(part 1 of 3)
# Autodesk Inventor assembly: 000 Ensamblaje hw_LM - BASIC
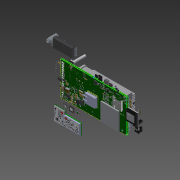
[picture p0: Inventor's stored thumbnail of the model, 180x180]
Saved by Autodesk Inventor 2018 (Build 220112000, 112)
## iProperties
Created: 2025-09-15
Part Number: 000 Ensamblaje hw_LM - BASIC
Document SubType Name: Assembly
Designer: mbs18
Author: mbs18
## Documents named in this file (68)
- C:\Users\mbs18.Embention\Git\LM\items\3d_LM\hw_LM\3d\000 Ensamblaje hw_LM - BASIC.iam
- C:\Users\mbs18.Embention\Git\LM\items\3d_LM\hw_LM\3d\hw_LM - PCB.ipt
- C:\Users\mbs18.Embention\Git\LM\items\_accesories\Cables y conectores\3d_Te Connectivity\3d\2309413-1\2309413-1.ipt
- C:\Users\mbs18.Embention\Git\LM\items\_accesories\Componentes PCB\Jetson Orin Nano\Nvidia\Jetson_Orin_NX_Orin_Nano_Module_3D_STEP_Model_20230310\P3767-pcba-envelop_20230310.ipt
- C:\Users\mbs18.Embention\Git\LM\items\_accesories\Componentes PCB\Tarjetero\3d_Molex\3d\47219-2001.ipt
- C:\Users\mbs18.Embention\Git\LM\items\_accesories\Componentes PCB\Magnetometro\3d_PNI Corp\3d\RM3100\Sen-XY-f.ipt
- C:\Users\mbs18.Embention\Git\LM\items\_accesories\Componentes PCB\Magnetometro\3d_PNI Corp\3d\RM3100\Sen-Z-f.ipt
- C:\Users\mbs18.Embention\Git\LM\items\_accesories\Componentes PCB\Transformadores de señal\3d_Pulse_Electronics\HX5008NL\HX5008NL.iam
- C:\Users\mbs18.Embention\Git\LM\items\_accesories\Componentes PCB\Conectores\3d_Samtec\3d\CLP-104-02-F-D-BE-TR.ipt
- C:\Users\mbs18.Embention\Git\LM\items\_accesories\Componentes PCB\Magnetometro\3d_PNI Corp\3d\RM3100\MAGI2C.ipt
- C:\Users\mbs18.Embention\Git\LM\items\_accesories\Componentes PCB\Inductor\3d_Vishay\IHLP2020CZER2R2MA1\IHLP2020CZER1R0M01.ipt
- C:\Users\mbs18.Embention\Git\LM\items\_accesories\Componentes PCB\Capacitadores\3d_Kemet\3d\CL31B106KBK6PJE.ipt
- C:\Users\mbs18.Embention\Git\LM\items\_accesories\Componentes PCB\Resistencias\3d_Genérico\R0805.ipt
- C:\Users\mbs18.Embention\Git\LM\items\_accesories\Componentes PCB\Resistencias\3d_Mouser Electronics\3d\ERJ-U02F1601X\RES-1.6K_1%_0402.iam
- C:\Users\mbs18.Embention\Git\LM\items\_accesories\Componentes PCB\Conversores\CC-CC\3d_MuRata\3d\3d_MGJ1D121505MPC-R7\UND_0201CR___ _________.ipt
- C:\Users\mbs18.Embention\Git\LM\items\_accesories\Componentes PCB\Led\3d_ROHM EXCELED\3d\SML-D12V8WT86C.ipt
- C:\Users\mbs18.Embention\Git\LM\items\_accesories\Componentes PCB\IMU\3d_Bosch\3d\BMI088.ipt
- C:\Users\mbs18.Embention\Git\LM\items\_accesories\Componentes PCB\Reguladores\3d_Texas Instruments\3d\TPS7A5301QRGRRQ1\TPS7A5301QRGRRQ1.iam
- C:\Users\mbs18.Embention\Git\LM\items\_accesories\Componentes PCB\Ferrita\3d_Murata Electronics\3d\BLM21PG220SN1D.ipt
- C:\Users\mbs18.Embention\Git\LM\items\_accesories\Componentes PCB\Condensadores\3d_KEMET\3d\C0603C101K5GAC3190\C0603C101K5GAC3190.ipt
- C:\Users\mbs18.Embention\Git\LM\items\_accesories\Componentes PCB\Capacitadores\3d_Kemet\3d\C1206C152KGRACAUTO.ipt
- C:\Users\mbs18.Embention\Git\LM\items\_accesories\Componentes PCB\Diodos\3d_Littlefuse\3d\AQ24CANFD-02HTG.ipt
- C:\Users\mbs18.Embention\Git\LM\items\_accesories\Componentes PCB\Oscilador\3d_ECS_International\ECS-2520MVQ-250-CN-TR\ECS-2520MVQ-250-CN-TR.ipt
- C:\Users\mbs18.Embention\Git\LM\items\_accesories\Componentes PCB\Jetson Orin Nano\Nvidia\Jetson_Orin_Nano_DevKit_3D_STEP_Model\095-0180-000-TS1_ASM.iam
- C:\Users\mbs18.Embention\Git\LM\items\_accesories\Componentes PCB\Microcontroladores\S32E288ABCAAMJGT.ipt
- C:\Users\mbs18.Embention\Git\LM\items\_accesories\Componentes PCB\Transceptor\3d_Texas Instrument\3d\DP83867ERGZT\DP83867ERGZT.iam
- C:\Users\mbs18.Embention\Git\LM\items\_accesories\Componentes PCB\DC-DC\3d_Linear Technology\3d\LTC7103IUHE#PBF.ipt
- C:\Users\mbs18.Embention\Git\LM\items\_accesories\Componentes PCB\CAN\3d\3d_Texas_Instruments\TCAN1462VDRBRQ1\TCAN1462VDRBRQ1.iam
- C:\Users\mbs18.Embention\Git\LM\items\_accesories\Componentes PCB\Mosfet\3d_Vishay\3d\SQJ465EP-T1_GE3\SQJ465EP-T1_GE3.iam
- C:\Users\mbs18.Embention\Git\LM\items\_accesories\Componentes PCB\Capacitadores\3d_Kyocera\3d\KAM55CR72A106KV-C2220K-simpl.ipt
- C:\Users\mbs18.Embention\Git\LM\items\_accesories\Componentes PCB\Schottky Diodes\3d_STMicroelectronics\3d\STPS5H100AFY\STPS5H100AFY.ipt
- C:\Users\mbs18.Embention\Git\LM\items\_accesories\Componentes PCB\Diodos\3d_Bourns\3d\SMA6J64CA\SMA6J64CA.ipt
- C:\Users\mbs18.Embention\Git\LM\items\_accesories\Componentes PCB\Condensadores\3d_KEMET\3d\C1210C472KGRACAUTO\C1210C472KGRACAUTO.ipt
- C:\Users\mbs18.Embention\Git\LM\items\_accesories\Componentes PCB\Mosfet\3d_Infineon\3d\BSS123NH6327XTSA1\BSS123NH6327XTSA1.iam
- C:\Users\mbs18.Embention\Git\LM\items\_accesories\Componentes PCB\Diodos\3d_Vishay\3d\BZD27C10P-HE3-08.ipt
- C:\Users\mbs18.Embention\Git\LM\items\_accesories\Componentes PCB\Condensadores\3d_KEMET\3d\C0603C103K1RECAUTO\C0603C103K1RECAUTO.iam
- C:\Users\mbs18.Embention\Git\LM\items\_accesories\Componentes PCB\DC-DC\3d_Texas Instruments\3d\LM5146QRGYRQ1\LM5146QRGYRQ1.iam
- C:\Users\mbs18.Embention\Git\LM\items\_accesories\Componentes PCB\Bobinas\3d_COILCRAFT\3d\1812CAN-113NRC\1812CAN-113NRC.iam
- C:\Users\mbs18.Embention\Git\LM\items\_accesories\Componentes PCB\Diodos\3d_ST Microelectronics\HSP051-4M10\HSP051-4M10.ipt
- C:\Users\mbs18.Embention\Git\LM\items\_accesories\Componentes PCB\IMU\3d_Analog Devices\3d\ADIS16505-3BMLZ\ADIS16505-3BMLZ.ipt
- C:\Users\mbs18.Embention\Git\LM\items\_accesories\Componentes PCB\SIM\3d_EMNIFY\3d\ESIM 638037665970.ipt
- C:\Users\mbs18.Embention\Git\LM\items\_accesories\Componentes PCB\CAN\3d\Analog Devices\LTC2875MPDD#PBF.ipt
- C:\Users\mbs18.Embention\Git\LM\items\_accesories\Componentes PCB\Transceptor\3d_Texas Instrument\3d\UQFN-16.ipt
- C:\Users\mbs18.Embention\Git\LM\items\_accesories\Componentes PCB\Oscilador\3d_ECS_International\ECS-400-8-33Q-ADS-TR.ipt
- C:\Users\mbs18.Embention\Git\LM\items\_accesories\Componentes PCB\DC-DC\3d_Texas Instruments\3d\TPS3897ADRYT.ipt
- C:\Users\mbs18.Embention\Git\LM\items\_accesories\Componentes PCB\ESD Protection\3d_Nexperia\3d\PESD2CANFD27V-UX\PESD2CANFD27V-UX.iam
- C:\Users\mbs18.Embention\Git\LM\items\_accesories\Componentes PCB\Diodos\3d_Diodes Incorporated\3d\DMN2710UTQ-7\DMN2710UTQ-7.ipt
- C:\Users\mbs18.Embention\Git\LM\items\_accesories\Componentes PCB\Multiplexor\3d_TI\3d\SN74LVC1G08QDCKRQ1.ipt
- C:\Users\mbs18.Embention\Git\LM\items\_accesories\Cables y conectores\3d_Molex\3d\53398-0471.ipt
- C:\Users\mbs18.Embention\Git\LM\items\_accesories\Componentes PCB\Bobinas\3d_COILCRAFT\3d\XAL7030-472MEC\XAL7030-472MEC.iam
- C:\Users\mbs18.Embention\Git\LM\items\_accesories\Componentes PCB\Mosfet\3d_Vishay\3d\SQJ402EP-T1_GE3.ipt
- C:\Users\mbs18.Embention\Git\LM\items\_accesories\Componentes PCB\Resistencias\3d_Genérico\MMB02070B1007GB200.ipt
- C:\Users\mbs18.Embention\Git\LM\items\_accesories\Componentes PCB\Inductor\3d_TDK\3d\XAL4020-601MEC\XAL4020-601MEC.ipt
- C:\Users\mbs18.Embention\Git\LM\items\_accesories\Componentes PCB\Reguladores\3d_Analog\3d\LTC3310SIV#PBF.ipt
- C:\Users\mbs18.Embention\Git\LM\items\_accesories\Componentes PCB\Diodos\3d_Texas Instrument\3d\TPD4E05U06QDQARQ1.ipt
- C:\Users\mbs18.Embention\Git\LM\items\_accesories\Componentes PCB\Diodos\3d_Littlefuse\3d\AQ05C-01FTG\AQ05C-01FTG.ipt
- C:\Users\mbs18.Embention\Git\LM\items\_accesories\Componentes PCB\GSM\3d_U-blox\3d\Sara\SARA.iam
- C:\Users\mbs18.Embention\Git\LM\items\_accesories\Componentes PCB\GPS - GNSS\3d_U-blox\3d\ZED F9P\u-blox ZED-F9P.ipt
- C:\Users\mbs18.Embention\Git\LM\items\_accesories\Componentes PCB\Elementos mecanicos soldables\3d_Wurth Electronics\3d\9774065151.ipt
- C:\Users\mbs18.Embention\Git\LM\items\_accesories\Ordenadores y Tablets\3d_NVIDIA\3d\Orin nano\Heatsink\ATS-NVP-3281-C2-R0.ipt
- C:\Users\mbs18.Embention\Git\LM\items\_accesories\Componentes PCB\Elementos mecanicos soldables\3d_Wurth Electronics\3d\9774130960R.ipt
- C:\Users\mbs18.Embention\Git\LM\items\_accesories\Sensores\Sensor de presion\3d_Amphenol\3d\AUAV-L10D-M25125-RR-N.ipt
- C:\Users\mbs18.Embention\Git\LM\items\_accesories\Componentes PCB\Resistencias\3d_Genérico\RESC-1210.ipt
- C:\Users\mbs18.Embention\Git\LM\items\_accesories\Componentes PCB\Reguladores\3d_Analog\3d\LIB_LTC7103MPUHE#PBF\LTC7103MPUHE#PBF.ipt
- C:\Users\mbs18.Embention\Git\LM\items\_accesories\Componentes PCB\Active-low load\3d_Texas_Instruments\TPS22910AYZVR\Body.ipt
- C:\Users\mbs18.Embention\Git\LM\items\_accesories\Componentes PCB\Led\3d_Lumex\3d\LPA-C011301S.ipt
- C:\Users\mbs18.Embention\Git\LM\items\_accesories\Componentes PCB\Sensores de Presion\3d_TE Connectivity\3d\MS561101BA03-50.ipt
- C:\Users\mbs18.Embention\Git\LM\items\_accesories\Componentes PCB\Sensores de Presion\3d_Infineon\3d\DPS368XTSA1.ipt
## Components (484 placed, 67 different names)
1. hw_LM - PCB:1 — Mate:1, Flush:1, Flush:2, Mate:4, Mate:29, Angle:6, Mate:33, Mate:35, Mate:47, Mate:58, Mate:59, Mate:60, Mate:69, Mate:72, Mate:73, Mate:81, Mate:83, Mate:84, Mate:94, Mate:95, Mate:96, Mate:97, Mate:98, Angle:44, Mate:99, Mate:100, Mate:101, Mate:102, Angle:45, Mate:103, Mate:104, Mate:105, Mate:107, Mate:108, Mate:109, Mate:110, Mate:112, Mate:113, Mate:114, Mate:115, Mate:116, Mate:117, Mate:118, Angle:49, Angle:50, Mate:119, Mate:120, Mate:121, Angle:53, Mate:122, Mate:123, Mate:124, Mate:125, Mate:126, Mate:127, Mate:128, Mate:129, Mate:130, Mate:131, Mate:132, Angle:59, Mate:133, Mate:134, Angle:62, Mate:135, Angle:64, Mate:136, Angle:86, Mate:137, Mate:138, Mate:139, Mate:140, Angle:88, Mate:141, Mate:142, Mate:143, Mate:144, Mate:145, Tangent:1, Mate:146, Mate:147, Mate:148, Mate:149, Mate:150, Mate:151, Mate:152, Mate:153, Mate:154, Mate:155, Angle:91, Mate:158, Angle:134, Angle:135, Mate:159, Mate:163, Mate:165, Mate:167, Mate:182, Mate:184, Mate:185, Mate:186, Mate:187, Mate:188, Mate:189, Mate:190, Mate:191, Mate:192, Mate:193
2. 095-0180-000-TS1_ASM:1 [sub-assembly]
3. 2309413-1:1 — Mate:4, Mate:58, Mate:59
4. P3767-pcba-envelop_20230310:1 — Mate:154, Mate:155, Mate:163, Mate:164, Mate:166, Mate:168, Mate:169, Mate:170, Mate:171
5. 47219-2001:1 — Mate:29, Angle:6
6. Sen-XY-f:1 — Mate:35, Flush:16
7. Sen-Z-f:1 — Mate:33
8. Sen-XY-f:2 — Flush:16
9. CLP-104-02-F-D-BE-TR:1 — Mate:47
10. HX5008NL:3 [sub-assembly] — Mate:83
11. HX5008NL:4 [sub-assembly] — Angle:44, Mate:99
12. MAGI2C:1 — Mate:60
13. IHLP2020CZER1R0M01:2
14. R0805:1 — Mate:69, Flush:39, Flush:40
15. R0805:2 — Flush:39
16. R0805:3 — Flush:40
17. CL31B106KBK6PJE:7 — Flush:43
18. CL31B106KBK6PJE:8 — Flush:43
19. UND_0201CR___ _________:1 — Mate:73, Flush:44
20. UND_0201CR___ _________:2 — Flush:44
21. BLM21PG220SN1D:4
22. C0603C101K5GAC3190:6 — Flush:119, Angle:56
23. C0603C101K5GAC3190:7 — Flush:119, Angle:56
24. BLM21PG220SN1D:11
25. C1206C152KGRACAUTO:1 — Mate:81, Flush:124, Angle:49
26. C1206C152KGRACAUTO:2 — Flush:123, Flush:124, Angle:48
27. C1206C152KGRACAUTO:3 — Flush:122, Flush:123, Flush:221, Flush:222, Flush:432
28. C1206C152KGRACAUTO:4 — Flush:122, Angle:48
29. BLM21PG220SN1D:12 — Flush:125
30. BLM21PG220SN1D:13 — Flush:125, Flush:126
31. BLM21PG220SN1D:14 — Flush:126, Flush:127
32. BLM21PG220SN1D:15 — Flush:127
33. AQ24CANFD-02HTG:5
34. AQ24CANFD-02HTG:6
35. AQ24CANFD-02HTG:7
36. AQ24CANFD-02HTG:8
37. S32E288ABCAAMJGT:1 — Mate:94, Angle:58, Angle:60, Angle:141
38. DP83867ERGZT:1 [sub-assembly] — Mate:95, Angle:43
39. ECS-2520MVQ-250-CN-TR:2 — Mate:96, Angle:43
40. LTC7103IUHE#PBF:1 — Mate:97
41. TCAN1462VDRBRQ1:1 [sub-assembly] — Mate:98, Flush:201
42. TCAN1462VDRBRQ1:2 [sub-assembly] — Flush:200
43. TCAN1462VDRBRQ1:3 [sub-assembly] — Flush:200, Flush:201
44. SQJ465EP-T1_GE3:1 [sub-assembly] — Mate:100, Mate:101
45. KAM55CR72A106KV-C2220K-simpl:1 — Mate:102, Angle:45, Angle:46, Angle:47
46. KAM55CR72A106KV-C2220K-simpl:2 — Mate:103, Angle:110
47. STPS5H100AFY:1 — Mate:104, Angle:46
48. STPS5H100AFY:3 — Mate:105, Angle:109
49. SML-D12V8WT86C:2 — Mate:107, Flush:202, Flush:611
50. SML-D12V8WT86C:3 — Mate:108
51. SML-D12V8WT86C:4 — Mate:109
52. SML-D12V8WT86C:5 — Mate:110
53. SML-D12V8WT86C:6 — Flush:202
54. SMA6J64CA:1 — Mate:116, Angle:47, Angle:63
55. SMA6J64CA:2 — Mate:117
56. C1210C472KGRACAUTO:1 — Mate:118, Flush:211
57. C1210C472KGRACAUTO:2 — Flush:210, Flush:211
58. C1210C472KGRACAUTO:3 — Flush:210
59. BSS123NH6327XTSA1:1 [sub-assembly] — Angle:50, Mate:119
60. BZD27C10P-HE3-08:1 — Mate:120
61. C0603C103K1RECAUTO:1 [sub-assembly] — Mate:121, Flush:217, Flush:219, Flush:335
62. C0603C103K1RECAUTO:2 [sub-assembly] — Flush:213, Flush:214
63. C0603C103K1RECAUTO:3 [sub-assembly] — Flush:218
64. C0603C103K1RECAUTO:4 [sub-assembly] — Flush:215
65. C0603C103K1RECAUTO:5 [sub-assembly] — Flush:212, Flush:213, Flush:216, Flush:217
66. C0603C103K1RECAUTO:6 [sub-assembly] — Flush:212, Flush:215, Flush:337
67. C0603C103K1RECAUTO:7 [sub-assembly] — Flush:214, Flush:427
68. C0603C103K1RECAUTO:8 [sub-assembly] — Flush:216, Flush:218, Flush:219
69. C0603C103K1RECAUTO:9 [sub-assembly] — Angle:53, Flush:222, Flush:223
70. C0603C103K1RECAUTO:10 [sub-assembly] — Flush:221
71. C0603C103K1RECAUTO:11 [sub-assembly] — Flush:223
72. C1210C472KGRACAUTO:7 — Flush:224
73. C1210C472KGRACAUTO:8 — Flush:224, Flush:231
74. LM5146QRGYRQ1:1 [sub-assembly] — Mate:122, Angle:76
75. 1812CAN-113NRC:1 [sub-assembly] — Mate:123
76. TCAN1462VDRBRQ1:5 [sub-assembly] — Mate:124
77. C1210C472KGRACAUTO:9 — Flush:229, Flush:231
78. C1210C472KGRACAUTO:10 — Flush:229
79. C1210C472KGRACAUTO:11 — Flush:228, Flush:230, Flush:232
80. C1210C472KGRACAUTO:12 — Flush:228, Flush:230, Flush:232, Angle:65
81. HSP051-4M10:1 — Mate:126, Flush:330, Flush:332
82. HSP051-4M10:2 — Flush:330
83. ADIS16505-3BMLZ:1 — Mate:127
84. BMI088:2 — Mate:128
85. ESIM 638037665970:1 — Mate:129, Angle:58
86. TPS7A5301QRGRRQ1:2 [sub-assembly] — Mate:130
87. LTC2875MPDD#PBF:1 — Mate:131, Flush:331
88. UQFN-16:1 — Mate:132, Angle:59
89. LTC2875MPDD#PBF:2 — Flush:331
90. ECS-400-8-33Q-ADS-TR:1 — Mate:133, Angle:60
91. TPS3897ADRYT:1 — Mate:134
92. HSP051-4M10:3 — Flush:332
93. PESD2CANFD27V-UX:1 [sub-assembly] — Angle:62, Mate:135, Angle:63
94. DMN2710UTQ-7:1 — Angle:64, Mate:136, Angle:65, Flush:333
95. DMN2710UTQ-7:2 — Flush:333, Flush:338
96. C0603C103K1RECAUTO:12 [sub-assembly] — Flush:334
97. C0603C103K1RECAUTO:13 [sub-assembly] — Flush:334, Flush:335
98. C0603C103K1RECAUTO:14 [sub-assembly] — Flush:336, Flush:337
99. C0603C103K1RECAUTO:15 [sub-assembly] — Flush:336
100. DMN2710UTQ-7:3 — Flush:339, Flush:340
101. DMN2710UTQ-7:4 — Flush:338, Flush:339, Flush:422
102. DMN2710UTQ-7:5 — Flush:340
103. DMN2710UTQ-7:6 — Flush:601
104. DMN2710UTQ-7:7 — Flush:422, Flush:423, Flush:603
105. DMN2710UTQ-7:8 — Flush:423
106. SN74LVC1G08QDCKRQ1:1 — Angle:86, Mate:137, Flush:602
107. C0603C103K1RECAUTO:16 [sub-assembly] — Flush:424, Flush:426, Flush:427
108. C0603C103K1RECAUTO:17 [sub-assembly] — Flush:425, Flush:426, Flush:431
109. C0603C103K1RECAUTO:18 [sub-assembly] — Flush:424
110. C0603C103K1RECAUTO:19 [sub-assembly] — Flush:425
111. C0603C103K1RECAUTO:20 [sub-assembly]
112. C0603C103K1RECAUTO:21 [sub-assembly] — Flush:431
113. C0603C103K1RECAUTO:22 [sub-assembly]
114. C0603C103K1RECAUTO:23 [sub-assembly]
115. UQFN-16:2 — Mate:138, Angle:141
116. C1206C152KGRACAUTO:5 — Flush:432
117. 53398-0471:1 — Mate:140, Angle:88
118. XAL7030-472MEC:1 [sub-assembly] — Mate:141, Flush:433
119. XAL7030-472MEC:2 [sub-assembly] — Flush:433
120. SQJ402EP-T1_GE3:1 — Mate:142, Mate:143
121. SQJ402EP-T1_GE3:2 — Mate:144, Mate:145
122. MMB02070B1007GB200:1 — Tangent:1
123. C1210C472KGRACAUTO:13 — Mate:146
124. C1206C152KGRACAUTO:6 — Mate:147
125. C1206C152KGRACAUTO:7 — Flush:436
126. C1206C152KGRACAUTO:8 — Flush:436
127. R0805:4 — Mate:148, Flush:437, Flush:440, Flush:443
128. R0805:5 — Flush:438, Flush:439
129. R0805:6 — Flush:439, Flush:440
130. R0805:7 — Flush:437, Flush:438
131. R0805:8
132. R0805:9
133. R0805:10 — Flush:443
134. 1812CAN-113NRC:2 [sub-assembly] — Mate:149
135. XAL4020-601MEC:1 — Mate:150, Flush:444
136. XAL4020-601MEC:2 — Flush:444
137. XAL4020-601MEC:3 — Mate:188
138. BZD27C10P-HE3-08:2 — Mate:151
139. LTC3310SIV#PBF:1 — Mate:152, Flush:446
140. LTC3310SIV#PBF:2 — Flush:446
141. TPD4E05U06QDQARQ1:1 — Mate:153, Flush:447
142. TPD4E05U06QDQARQ1:2 — Flush:448
143. TPD4E05U06QDQARQ1:3 — Flush:447, Flush:448
144. PESD2CANFD27V-UX:2 [sub-assembly] — Mate:158, Angle:109, Flush:536
145. PESD2CANFD27V-UX:3 [sub-assembly] — Flush:536, Angle:110
146. AQ05C-01FTG:1 — Angle:134, Angle:135, Mate:159
147. u-blox ZED-F9P:1 — Mate:185, Angle:137
148. 9774065151:1 — Mate:164, Mate:165
149. 9774065151:2 — Mate:166, Mate:167
150. ATS-NVP-3281-C2-R0:1 — Mate:168, Mate:169, Mate:170, Mate:171
151. AUAV-L10D-M25125-RR-N:1 — Mate:182, Angle:139
152. SARA:1 [sub-assembly] — Mate:184, Angle:138
153. DMN2710UTQ-7:9 — Flush:601
154. SN74LVC1G08QDCKRQ1:2 — Flush:602
155. DMN2710UTQ-7:10 — Flush:603
156. RESC-1210:1 — Mate:186, Angle:137
157. LTC7103MPUHE#PBF:1 — Mate:187, Angle:138
158. C1210C472KGRACAUTO:14 — Mate:189, Angle:139, Flush:605, Flush:609
159. C1210C472KGRACAUTO:15 — Flush:604, Flush:605, Flush:608
160. C1210C472KGRACAUTO:16 — Flush:604, Flush:606, Flush:607
161. C1210C472KGRACAUTO:17 — Flush:606, Flush:608
162. C1210C472KGRACAUTO:18 — Flush:607
163. C1210C472KGRACAUTO:19
164. C1210C472KGRACAUTO:20 — Flush:610
165. C1210C472KGRACAUTO:21 — Flush:609, Flush:610
166. Body:1 — Mate:190
167. LPA-C011301S:1 — Mate:191
168. SML-D12V8WT86C:7 — Flush:611
169. MS561101BA03-50:1 — Mate:192, Angle:140
170. DPS368XTSA1:1 — Mate:193
171. 9774130960R:1
172. RES-1.6K_1%_0402:263 [sub-assembly] — Angle:95, Flush:517, Flush:535
173. RES-1.6K_1%_0402:1 [sub-assembly] — Mate:72
174. RES-1.6K_1%_0402:7 [sub-assembly] — Flush:58, Flush:63, Flush:68
175. RES-1.6K_1%_0402:8 [sub-assembly] — Flush:58, Flush:59
176. RES-1.6K_1%_0402:9 [sub-assembly] — Flush:59, Flush:245, Flush:253
177. RES-1.6K_1%_0402:10 [sub-assembly]
178. RES-1.6K_1%_0402:11 [sub-assembly] — Flush:63
179. RES-1.6K_1%_0402:12 [sub-assembly] — Flush:67
180. RES-1.6K_1%_0402:13 [sub-assembly] — Flush:66, Flush:67, Flush:68
181. RES-1.6K_1%_0402:14 [sub-assembly] — Flush:64, Flush:65
182. RES-1.6K_1%_0402:15 [sub-assembly] — Flush:65, Flush:66
183. RES-1.6K_1%_0402:16 [sub-assembly] — Flush:64, Flush:73, Flush:87, Flush:118
184. RES-1.6K_1%_0402:17 [sub-assembly]
185. RES-1.6K_1%_0402:18 [sub-assembly] — Flush:73
186. RES-1.6K_1%_0402:19 [sub-assembly]
187. RES-1.6K_1%_0402:20 [sub-assembly]
188. RES-1.6K_1%_0402:21 [sub-assembly]
189. RES-1.6K_1%_0402:22 [sub-assembly] — Flush:85, Flush:86
190. RES-1.6K_1%_0402:23 [sub-assembly] — Flush:87, Flush:142
191. RES-1.6K_1%_0402:24 [sub-assembly] — Flush:84
192. RES-1.6K_1%_0402:25 [sub-assembly]
193. RES-1.6K_1%_0402:26 [sub-assembly] — Flush:88
194. RES-1.6K_1%_0402:27 [sub-assembly] — Flush:84, Flush:85
195. RES-1.6K_1%_0402:28 [sub-assembly]
196. RES-1.6K_1%_0402:29 [sub-assembly] — Flush:86
197. RES-1.6K_1%_0402:30 [sub-assembly] — Flush:89, Flush:198
198. RES-1.6K_1%_0402:31 [sub-assembly] — Flush:88, Flush:89, Flush:109, Flush:420
199. RES-1.6K_1%_0402:32 [sub-assembly]
200. RES-1.6K_1%_0402:34 [sub-assembly]
201. RES-1.6K_1%_0402:35 [sub-assembly]
202. RES-1.6K_1%_0402:36 [sub-assembly] — Flush:109
203. RES-1.6K_1%_0402:38 [sub-assembly]
204. RES-1.6K_1%_0402:39 [sub-assembly]
205. RES-1.6K_1%_0402:40 [sub-assembly] — Flush:118, Flush:121
206. RES-1.6K_1%_0402:41 [sub-assembly]
207. RES-1.6K_1%_0402:42 [sub-assembly]
208. RES-1.6K_1%_0402:43 [sub-assembly] — Flush:121
209. RES-1.6K_1%_0402:44 [sub-assembly] — Flush:138, Flush:155
210. RES-1.6K_1%_0402:45 [sub-assembly] — Flush:156
211. RES-1.6K_1%_0402:46 [sub-assembly] — Flush:155
212. RES-1.6K_1%_0402:47 [sub-assembly] — Flush:142, Flush:158
213. RES-1.6K_1%_0402:48 [sub-assembly] — Flush:143
214. RES-1.6K_1%_0402:49 [sub-assembly] — Flush:152
215. RES-1.6K_1%_0402:50 [sub-assembly] — Flush:153
216. RES-1.6K_1%_0402:51 [sub-assembly] — Flush:153, Flush:154
217. RES-1.6K_1%_0402:52 [sub-assembly] — Flush:139, Flush:148, Flush:152
218. RES-1.6K_1%_0402:53 [sub-assembly] — Flush:148
219. RES-1.6K_1%_0402:54 [sub-assembly] — Flush:149
220. RES-1.6K_1%_0402:55 [sub-assembly] — Flush:137, Flush:145, Flush:147, Flush:149, Flush:150, Flush:154, Flush:156
221. RES-1.6K_1%_0402:56 [sub-assembly] — Flush:138, Mate:84, Flush:144, Flush:146, Flush:151
222. RES-1.6K_1%_0402:57 [sub-assembly] — Flush:143, Flush:144
223. RES-1.6K_1%_0402:58 [sub-assembly] — Flush:146
224. RES-1.6K_1%_0402:59 [sub-assembly] — Flush:137, Flush:139, Flush:145, Flush:147, Flush:150, Flush:151
225. RES-1.6K_1%_0402:60 [sub-assembly] — Flush:159
226. RES-1.6K_1%_0402:61 [sub-assembly] — Flush:160
227. RES-1.6K_1%_0402:62 [sub-assembly] — Flush:164, Flush:168
228. RES-1.6K_1%_0402:63 [sub-assembly] — Flush:158, Flush:159, Flush:160, Flush:175
229. RES-1.6K_1%_0402:64 [sub-assembly]
230. RES-1.6K_1%_0402:65 [sub-assembly] — Flush:164
231. RES-1.6K_1%_0402:66 [sub-assembly] — Flush:183
232. RES-1.6K_1%_0402:67 [sub-assembly] — Flush:182
233. RES-1.6K_1%_0402:68 [sub-assembly]
234. RES-1.6K_1%_0402:69 [sub-assembly] — Flush:168
235. RES-1.6K_1%_0402:70 [sub-assembly]
236. RES-1.6K_1%_0402:71 [sub-assembly]
237. RES-1.6K_1%_0402:72 [sub-assembly] — Flush:174
238. RES-1.6K_1%_0402:73 [sub-assembly]
239. RES-1.6K_1%_0402:74 [sub-assembly] — Flush:175
240. RES-1.6K_1%_0402:75 [sub-assembly] — Flush:174
241. RES-1.6K_1%_0402:76 [sub-assembly] — Flush:183
242. RES-1.6K_1%_0402:77 [sub-assembly]
243. RES-1.6K_1%_0402:78 [sub-assembly] — Flush:186
244. RES-1.6K_1%_0402:79 [sub-assembly] — Flush:182
245. RES-1.6K_1%_0402:80 [sub-assembly] — Flush:186
246. RES-1.6K_1%_0402:81 [sub-assembly]
247. RES-1.6K_1%_0402:82 [sub-assembly] — Flush:190
248. RES-1.6K_1%_0402:83 [sub-assembly] — Flush:190, Flush:191
249. RES-1.6K_1%_0402:84 [sub-assembly] — Flush:191, Flush:192
250. RES-1.6K_1%_0402:85 [sub-assembly] — Flush:192, Flush:194, Flush:246
251. RES-1.6K_1%_0402:86 [sub-assembly] — Flush:194
252. RES-1.6K_1%_0402:87 [sub-assembly] — Flush:197, Flush:198
253. RES-1.6K_1%_0402:88 [sub-assembly] — Flush:197
254. RES-1.6K_1%_0402:89 [sub-assembly] — Mate:115, Flush:204, Flush:205
255. RES-1.6K_1%_0402:90 [sub-assembly] — Mate:114, Flush:205, Flush:206
256. RES-1.6K_1%_0402:91 [sub-assembly] — Mate:113, Flush:206, Flush:207
257. RES-1.6K_1%_0402:92 [sub-assembly] — Mate:112, Flush:207
258. RES-1.6K_1%_0402:94 [sub-assembly] — Flush:204
259. RES-1.6K_1%_0402:95 [sub-assembly]
260. RES-1.6K_1%_0402:96 [sub-assembly]
261. RES-1.6K_1%_0402:97 [sub-assembly] — Mate:139, Flush:451, Flush:467, Flush:479, Flush:492, Flush:518
262. RES-1.6K_1%_0402:98 [sub-assembly] — Flush:242, Flush:245
263. RES-1.6K_1%_0402:99 [sub-assembly] — Flush:242, Flush:243
264. RES-1.6K_1%_0402:100 [sub-assembly] — Flush:240, Flush:243, Mate:125, Flush:329
265. RES-1.6K_1%_0402:101 [sub-assembly] — Flush:241, Flush:244
266. RES-1.6K_1%_0402:102 [sub-assembly] — Flush:240, Flush:246
267. RES-1.6K_1%_0402:103 [sub-assembly] — Flush:241, Flush:244
268. RES-1.6K_1%_0402:104 [sub-assembly] — Flush:251
269. RES-1.6K_1%_0402:105 [sub-assembly] — Flush:252, Flush:261, Flush:278
270. RES-1.6K_1%_0402:106 [sub-assembly] — Flush:250, Flush:253
271. RES-1.6K_1%_0402:107 [sub-assembly] — Flush:249, Flush:252, Flush:260
272. RES-1.6K_1%_0402:108 [sub-assembly] — Flush:250
273. RES-1.6K_1%_0402:109 [sub-assembly] — Flush:249, Flush:251
274. RES-1.6K_1%_0402:110 [sub-assembly]
275. RES-1.6K_1%_0402:111 [sub-assembly]
276. RES-1.6K_1%_0402:112 [sub-assembly] — Flush:260
277. RES-1.6K_1%_0402:113 [sub-assembly] — Flush:261, Flush:296, Flush:319
278. RES-1.6K_1%_0402:114 [sub-assembly]
279. RES-1.6K_1%_0402:115 [sub-assembly] — Flush:276
280. RES-1.6K_1%_0402:116 [sub-assembly]
281. RES-1.6K_1%_0402:117 [sub-assembly] — Flush:295
282. RES-1.6K_1%_0402:118 [sub-assembly]
283. RES-1.6K_1%_0402:119 [sub-assembly]
284. RES-1.6K_1%_0402:120 [sub-assembly] — Flush:277, Flush:278
285. RES-1.6K_1%_0402:121 [sub-assembly]
286. RES-1.6K_1%_0402:122 [sub-assembly] — Flush:276
287. RES-1.6K_1%_0402:123 [sub-assembly]
288. RES-1.6K_1%_0402:124 [sub-assembly]
289. RES-1.6K_1%_0402:125 [sub-assembly]
290. RES-1.6K_1%_0402:126 [sub-assembly] — Flush:277
291. RES-1.6K_1%_0402:127 [sub-assembly]
292. RES-1.6K_1%_0402:128 [sub-assembly]
293. RES-1.6K_1%_0402:129 [sub-assembly]
294. RES-1.6K_1%_0402:130 [sub-assembly]
295. RES-1.6K_1%_0402:131 [sub-assembly]
296. RES-1.6K_1%_0402:132 [sub-assembly]
297. RES-1.6K_1%_0402:133 [sub-assembly]
298. RES-1.6K_1%_0402:134 [sub-assembly] — Flush:294
299. RES-1.6K_1%_0402:135 [sub-assembly]
300. RES-1.6K_1%_0402:136 [sub-assembly]
301. RES-1.6K_1%_0402:137 [sub-assembly] — Flush:296
302. RES-1.6K_1%_0402:138 [sub-assembly]
303. RES-1.6K_1%_0402:139 [sub-assembly] — Flush:294, Flush:295
304. RES-1.6K_1%_0402:140 [sub-assembly]
305. RES-1.6K_1%_0402:141 [sub-assembly]
306. RES-1.6K_1%_0402:142 [sub-assembly] — Flush:329, Flush:344
307. RES-1.6K_1%_0402:143 [sub-assembly] — Flush:327, Flush:345, Flush:353
308. RES-1.6K_1%_0402:144 [sub-assembly] — Flush:324
309. RES-1.6K_1%_0402:145 [sub-assembly] — Flush:317, Flush:323, Flush:328
310. RES-1.6K_1%_0402:146 [sub-assembly] — Flush:326, Flush:346, Flush:354
311. RES-1.6K_1%_0402:147 [sub-assembly] — Flush:318
312. RES-1.6K_1%_0402:148 [sub-assembly]
313. RES-1.6K_1%_0402:149 [sub-assembly]
314. RES-1.6K_1%_0402:150 [sub-assembly] — Flush:319
315. RES-1.6K_1%_0402:151 [sub-assembly]
316. RES-1.6K_1%_0402:152 [sub-assembly]
317. RES-1.6K_1%_0402:153 [sub-assembly]
318. RES-1.6K_1%_0402:154 [sub-assembly]
319. RES-1.6K_1%_0402:155 [sub-assembly] — Flush:318
320. RES-1.6K_1%_0402:156 [sub-assembly]
321. RES-1.6K_1%_0402:157 [sub-assembly] — Flush:317
322. RES-1.6K_1%_0402:158 [sub-assembly]
323. RES-1.6K_1%_0402:159 [sub-assembly]
324. RES-1.6K_1%_0402:160 [sub-assembly] — Flush:326
325. RES-1.6K_1%_0402:161 [sub-assembly] — Flush:324, Flush:325, Flush:328
326. RES-1.6K_1%_0402:162 [sub-assembly] — Flush:325
327. RES-1.6K_1%_0402:163 [sub-assembly] — Flush:323
328. RES-1.6K_1%_0402:164 [sub-assembly] — Flush:327
329. RES-1.6K_1%_0402:165 [sub-assembly] — Flush:345
330. RES-1.6K_1%_0402:166 [sub-assembly]
331. RES-1.6K_1%_0402:167 [sub-assembly] — Flush:344
332. RES-1.6K_1%_0402:168 [sub-assembly] — Flush:346
333. RES-1.6K_1%_0402:170 [sub-assembly] — Flush:355, Flush:382
334. RES-1.6K_1%_0402:171 [sub-assembly] — Flush:356
335. RES-1.6K_1%_0402:172 [sub-assembly]
336. RES-1.6K_1%_0402:173 [sub-assembly]
337. RES-1.6K_1%_0402:174 [sub-assembly] — Flush:381
338. RES-1.6K_1%_0402:175 [sub-assembly] — Flush:354
339. RES-1.6K_1%_0402:176 [sub-assembly] — Flush:355
340. RES-1.6K_1%_0402:177 [sub-assembly] — Flush:353, Flush:356
341. RES-1.6K_1%_0402:178 [sub-assembly]
342. RES-1.6K_1%_0402:179 [sub-assembly]
343. RES-1.6K_1%_0402:180 [sub-assembly]
344. RES-1.6K_1%_0402:181 [sub-assembly]
345. RES-1.6K_1%_0402:182 [sub-assembly] — Flush:381
346. RES-1.6K_1%_0402:183 [sub-assembly] — Flush:382, Flush:383
347. RES-1.6K_1%_0402:184 [sub-assembly]
348. RES-1.6K_1%_0402:185 [sub-assembly] — Flush:384
349. RES-1.6K_1%_0402:186 [sub-assembly] — Angle:73, Angle:74, Flush:399
350. RES-1.6K_1%_0402:187 [sub-assembly] — Flush:386, Angle:74
351. RES-1.6K_1%_0402:188 [sub-assembly] — Flush:387, Angle:75
352. RES-1.6K_1%_0402:189 [sub-assembly] — Flush:388, Angle:71, Angle:72, Angle:75
353. RES-1.6K_1%_0402:190 [sub-assembly] — Flush:385, Angle:70, Angle:71
354. RES-1.6K_1%_0402:191 [sub-assembly] — Angle:69, Angle:70, Flush:398
355. RES-1.6K_1%_0402:192 [sub-assembly] — Angle:69, Angle:76
356. RES-1.6K_1%_0402:193 [sub-assembly] — Angle:72, Angle:73, Flush:397
357. RES-1.6K_1%_0402:194 [sub-assembly]
358. RES-1.6K_1%_0402:195 [sub-assembly]
359. RES-1.6K_1%_0402:196 [sub-assembly]
360. RES-1.6K_1%_0402:197 [sub-assembly] — Flush:386
361. RES-1.6K_1%_0402:198 [sub-assembly] — Flush:383
362. RES-1.6K_1%_0402:199 [sub-assembly] — Flush:385
363. RES-1.6K_1%_0402:200 [sub-assembly] — Flush:384, Flush:388
364. RES-1.6K_1%_0402:201 [sub-assembly] — Flush:387
365. RES-1.6K_1%_0402:202 [sub-assembly] — Flush:398
366. RES-1.6K_1%_0402:203 [sub-assembly]
367. RES-1.6K_1%_0402:204 [sub-assembly] — Flush:397
368. RES-1.6K_1%_0402:205 [sub-assembly]
369. RES-1.6K_1%_0402:206 [sub-assembly] — Flush:399
370. RES-1.6K_1%_0402:207 [sub-assembly]
371. RES-1.6K_1%_0402:208 [sub-assembly]
372. RES-1.6K_1%_0402:209 [sub-assembly]
373. RES-1.6K_1%_0402:210 [sub-assembly] — Flush:413, Flush:419
374. RES-1.6K_1%_0402:211 [sub-assembly]
375. RES-1.6K_1%_0402:212 [sub-assembly]
376. RES-1.6K_1%_0402:213 [sub-assembly] — Flush:416
377. RES-1.6K_1%_0402:214 [sub-assembly] — Flush:418
378. RES-1.6K_1%_0402:215 [sub-assembly] — Flush:412, Flush:417
379. RES-1.6K_1%_0402:216 [sub-assembly] — Flush:414
380. RES-1.6K_1%_0402:217 [sub-assembly] — Flush:414, Flush:418, Flush:419
381. RES-1.6K_1%_0402:218 [sub-assembly]
382. RES-1.6K_1%_0402:219 [sub-assembly] — Flush:413
383. RES-1.6K_1%_0402:220 [sub-assembly] — Flush:412, Flush:415, Flush:420
384. RES-1.6K_1%_0402:221 [sub-assembly] — Flush:417
385. RES-1.6K_1%_0402:222 [sub-assembly] — Flush:415
386. RES-1.6K_1%_0402:223 [sub-assembly] — Flush:416
387. RES-1.6K_1%_0402:224 [sub-assembly] — Flush:452, Flush:466
388. RES-1.6K_1%_0402:225 [sub-assembly] — Flush:453, Flush:454, Flush:463, Flush:595
389. RES-1.6K_1%_0402:226 [sub-assembly] — Flush:450, Flush:451, Flush:452, Flush:453, Flush:467, Flush:476
390. RES-1.6K_1%_0402:227 [sub-assembly] — Flush:450, Flush:454
391. RES-1.6K_1%_0402:228 [sub-assembly] — Flush:465
392. RES-1.6K_1%_0402:229 [sub-assembly] — Flush:464
393. RES-1.6K_1%_0402:230 [sub-assembly] — Flush:463
394. RES-1.6K_1%_0402:231 [sub-assembly]
395. RES-1.6K_1%_0402:232 [sub-assembly] — Flush:464, Flush:477
396. RES-1.6K_1%_0402:233 [sub-assembly] — Flush:465
397. RES-1.6K_1%_0402:234 [sub-assembly] — Flush:479, Flush:480
398. RES-1.6K_1%_0402:235 [sub-assembly] — Flush:466
399. RES-1.6K_1%_0402:236 [sub-assembly] — Flush:478
400. RES-1.6K_1%_0402:237 [sub-assembly] — Flush:477
401. RES-1.6K_1%_0402:238 [sub-assembly]
402. RES-1.6K_1%_0402:239 [sub-assembly] — Flush:476
403. RES-1.6K_1%_0402:240 [sub-assembly] — Flush:480
404. RES-1.6K_1%_0402:241 [sub-assembly] — Flush:478
405. RES-1.6K_1%_0402:242 [sub-assembly] — Flush:489
406. RES-1.6K_1%_0402:243 [sub-assembly]
407. RES-1.6K_1%_0402:244 [sub-assembly]
408. RES-1.6K_1%_0402:245 [sub-assembly]
409. RES-1.6K_1%_0402:246 [sub-assembly] — Flush:489, Flush:490
410. RES-1.6K_1%_0402:247 [sub-assembly] — Flush:491
411. RES-1.6K_1%_0402:248 [sub-assembly] — Flush:490, Flush:503
412. RES-1.6K_1%_0402:249 [sub-assembly] — Flush:491, Flush:492
413. RES-1.6K_1%_0402:250 [sub-assembly]
414. RES-1.6K_1%_0402:251 [sub-assembly] — Flush:501
415. RES-1.6K_1%_0402:252 [sub-assembly]
416. RES-1.6K_1%_0402:253 [sub-assembly] — Flush:502, Flush:504
417. RES-1.6K_1%_0402:254 [sub-assembly]
418. RES-1.6K_1%_0402:255 [sub-assembly] — Flush:501
419. RES-1.6K_1%_0402:256 [sub-assembly] — Flush:504
420. RES-1.6K_1%_0402:257 [sub-assembly] — Angle:93, Angle:94, Angle:97
421. RES-1.6K_1%_0402:258 [sub-assembly] — Flush:503, Angle:91, Angle:92, Angle:93, Flush:550, Flush:551
422. RES-1.6K_1%_0402:259 [sub-assembly] — Flush:502, Angle:92, Flush:515
423. RES-1.6K_1%_0402:260 [sub-assembly] — Angle:97, Angle:98, Angle:99
424. RES-1.6K_1%_0402:261 [sub-assembly] — Angle:98
425. RES-1.6K_1%_0402:262 [sub-assembly] — Angle:99, Flush:595
426. RES-1.6K_1%_0402:264 [sub-assembly] — Angle:94, Angle:95, Angle:96
427. RES-1.6K_1%_0402:265 [sub-assembly] — Angle:96
428. RES-1.6K_1%_0402:266 [sub-assembly] — Flush:516
429. RES-1.6K_1%_0402:267 [sub-assembly] — Flush:516, Flush:517
430. RES-1.6K_1%_0402:268 [sub-assembly] — Flush:515, Flush:535
431. RES-1.6K_1%_0402:269 [sub-assembly]
432. RES-1.6K_1%_0402:270 [sub-assembly] — Flush:518
433. RES-1.6K_1%_0402:272 [sub-assembly] — Flush:532, Flush:534
434. RES-1.6K_1%_0402:273 [sub-assembly] — Flush:532, Flush:534
435. RES-1.6K_1%_0402:274 [sub-assembly]
436. RES-1.6K_1%_0402:275 [sub-assembly] — Flush:533
437. RES-1.6K_1%_0402:276 [sub-assembly]
438. RES-1.6K_1%_0402:277 [sub-assembly] — Flush:530
439. RES-1.6K_1%_0402:278 [sub-assembly] — Flush:530, Flush:533
440. RES-1.6K_1%_0402:279 [sub-assembly]
441. RES-1.6K_1%_0402:280 [sub-assembly] — Flush:546
442. RES-1.6K_1%_0402:282 [sub-assembly] — Flush:549, Flush:564, Flush:565
443. RES-1.6K_1%_0402:283 [sub-assembly] — Flush:545, Flush:546, Flush:550, Flush:571, Flush:584, Flush:589
444. RES-1.6K_1%_0402:284 [sub-assembly]
445. RES-1.6K_1%_0402:285 [sub-assembly] — Flush:547
446. RES-1.6K_1%_0402:286 [sub-assembly] — Flush:545, Flush:547, Flush:548, Flush:567
447. RES-1.6K_1%_0402:287 [sub-assembly] — Flush:549, Flush:551, Flush:570
448. RES-1.6K_1%_0402:288 [sub-assembly] — Flush:579, Flush:583, Flush:588
449. RES-1.6K_1%_0402:289 [sub-assembly] — Flush:548, Flush:566
450. RES-1.6K_1%_0402:290 [sub-assembly] — Flush:565, Angle:140
451. RES-1.6K_1%_0402:291 [sub-assembly] — Flush:566, Flush:594
452. RES-1.6K_1%_0402:292 [sub-assembly]
453. RES-1.6K_1%_0402:293 [sub-assembly] — Flush:567
454. RES-1.6K_1%_0402:294 [sub-assembly]
455. RES-1.6K_1%_0402:295 [sub-assembly]
456. RES-1.6K_1%_0402:296 [sub-assembly]
457. RES-1.6K_1%_0402:297 [sub-assembly] — Flush:564
458. RES-1.6K_1%_0402:298 [sub-assembly]
459. RES-1.6K_1%_0402:299 [sub-assembly] — Flush:571, Flush:578
460. RES-1.6K_1%_0402:300 [sub-assembly] — Flush:570
461. RES-1.6K_1%_0402:301 [sub-assembly] — Flush:577
462. RES-1.6K_1%_0402:302 [sub-assembly]
463. RES-1.6K_1%_0402:303 [sub-assembly] — Flush:580
464. RES-1.6K_1%_0402:304 [sub-assembly] — Flush:577
465. RES-1.6K_1%_0402:305 [sub-assembly] — Flush:578
466. RES-1.6K_1%_0402:306 [sub-assembly] — Flush:582, Flush:585, Flush:590
467. RES-1.6K_1%_0402:307 [sub-assembly] — Flush:579
468. RES-1.6K_1%_0402:308 [sub-assembly]
469. RES-1.6K_1%_0402:309 [sub-assembly] — Flush:594
470. RES-1.6K_1%_0402:310 [sub-assembly] — Flush:580
471. RES-1.6K_1%_0402:311 [sub-assembly] — Flush:585, Flush:596
472. RES-1.6K_1%_0402:312 [sub-assembly] — Flush:583, Flush:597
473. RES-1.6K_1%_0402:313 [sub-assembly] — Flush:584
474. RES-1.6K_1%_0402:314 [sub-assembly] — Flush:582
475. RES-1.6K_1%_0402:315 [sub-assembly] — Flush:597
476. RES-1.6K_1%_0402:316 [sub-assembly] — Flush:596
477. RES-1.6K_1%_0402:317 [sub-assembly] — Flush:588
478. RES-1.6K_1%_0402:318 [sub-assembly] — Flush:589
479. RES-1.6K_1%_0402:319 [sub-assembly]
480. RES-1.6K_1%_0402:320 [sub-assembly]
481. RES-1.6K_1%_0402:321 [sub-assembly] — Flush:590, Flush:593
482. RES-1.6K_1%_0402:322 [sub-assembly] — Flush:591, Flush:592
483. RES-1.6K_1%_0402:323 [sub-assembly] — Flush:592
484. RES-1.6K_1%_0402:324 [sub-assembly] — Flush:591, Flush:593
## Relationships (694: Flush 516, Mate 97, Angle 80, Tangent 1)
- Mate:1: hw_LM - PCB:1
- Flush:1: hw_LM - PCB:1
- Flush:2: hw_LM - PCB:1
- Mate:4: hw_LM - PCB:1 ↔ 2309413-1:1
- Mate:29: hw_LM - PCB:1 ↔ 47219-2001:1
- Angle:6 (180 deg): hw_LM - PCB:1 ↔ 47219-2001:1
- Mate:33: hw_LM - PCB:1 ↔ Sen-Z-f:1
- Mate:35: hw_LM - PCB:1 ↔ Sen-XY-f:1
- Flush:16: Sen-XY-f:1 ↔ Sen-XY-f:2
- Mate:47: hw_LM - PCB:1 ↔ CLP-104-02-F-D-BE-TR:1
- Mate:58: hw_LM - PCB:1 ↔ 2309413-1:1
- Mate:59: hw_LM - PCB:1 ↔ 2309413-1:1
- Mate:60: hw_LM - PCB:1 ↔ MAGI2C:1
- Mate:69: hw_LM - PCB:1 ↔ R0805:1
- Flush:39: R0805:1 ↔ R0805:2
- Flush:40: R0805:1 ↔ R0805:3
- Flush:43: CL31B106KBK6PJE:7 ↔ CL31B106KBK6PJE:8
- Mate:72: hw_LM - PCB:1 ↔ RES-1.6K_1%_0402:1
- Mate:73: hw_LM - PCB:1 ↔ UND_0201CR___ _________:1
- Flush:44: UND_0201CR___ _________:1 ↔ UND_0201CR___ _________:2
- [Flush]: RES-1.6K_1%_0402:7 ↔ RES-1.6K_1%_0402:9
- [Flush]: RES-1.6K_1%_0402:8 ↔ RES-1.6K_1%_0402:9
- Flush:58: RES-1.6K_1%_0402:7 ↔ RES-1.6K_1%_0402:8
- Flush:59: RES-1.6K_1%_0402:8 ↔ RES-1.6K_1%_0402:9
- [Flush]: RES-1.6K_1%_0402:10 ↔ RES-1.6K_1%_0402:11
- [Flush]: RES-1.6K_1%_0402:10 ↔ RES-1.6K_1%_0402:11
- Flush:63: RES-1.6K_1%_0402:7 ↔ RES-1.6K_1%_0402:11
- Flush:64: RES-1.6K_1%_0402:14 ↔ RES-1.6K_1%_0402:16
- Flush:65: RES-1.6K_1%_0402:14 ↔ RES-1.6K_1%_0402:15
- Flush:66: RES-1.6K_1%_0402:13 ↔ RES-1.6K_1%_0402:15
- Flush:67: RES-1.6K_1%_0402:12 ↔ RES-1.6K_1%_0402:13
- Flush:68: RES-1.6K_1%_0402:7 ↔ RES-1.6K_1%_0402:13
- [Flush]: RES-1.6K_1%_0402:19 ↔ RES-1.6K_1%_0402:21
- [Flush]: RES-1.6K_1%_0402:19 ↔ RES-1.6K_1%_0402:20
- [Flush]: RES-1.6K_1%_0402:18 ↔ RES-1.6K_1%_0402:20
- [Flush]: RES-1.6K_1%_0402:17 ↔ RES-1.6K_1%_0402:18
- Flush:73: RES-1.6K_1%_0402:16 ↔ RES-1.6K_1%_0402:18
- [Flush]: RES-1.6K_1%_0402:22 ↔ RES-1.6K_1%_0402:24
- [Flush]: RES-1.6K_1%_0402:23 ↔ RES-1.6K_1%_0402:24
- [Flush]: RES-1.6K_1%_0402:22 ↔ RES-1.6K_1%_0402:23
- [Flush]: RES-1.6K_1%_0402:23 ↔ RES-1.6K_1%_0402:24
- [Flush]: RES-1.6K_1%_0402:22 ↔ RES-1.6K_1%_0402:25
- [Flush]: RES-1.6K_1%_0402:26 ↔ RES-1.6K_1%_0402:28
- [Flush]: RES-1.6K_1%_0402:27 ↔ RES-1.6K_1%_0402:28
- [Flush]: RES-1.6K_1%_0402:26 ↔ RES-1.6K_1%_0402:27
- [Flush]: RES-1.6K_1%_0402:27 ↔ RES-1.6K_1%_0402:28
- [Flush]: RES-1.6K_1%_0402:26 ↔ RES-1.6K_1%_0402:29
- Flush:84: RES-1.6K_1%_0402:24 ↔ RES-1.6K_1%_0402:27
- Flush:85: RES-1.6K_1%_0402:22 ↔ RES-1.6K_1%_0402:27
- Flush:86: RES-1.6K_1%_0402:22 ↔ RES-1.6K_1%_0402:29
- Flush:87: RES-1.6K_1%_0402:16 ↔ RES-1.6K_1%_0402:23
- Flush:88: RES-1.6K_1%_0402:26 ↔ RES-1.6K_1%_0402:31
- Flush:89: RES-1.6K_1%_0402:30 ↔ RES-1.6K_1%_0402:31
- [Flush]: RES-1.6K_1%_0402:34 ↔ RES-1.6K_1%_0402:36
- [Flush]: RES-1.6K_1%_0402:34 ↔ RES-1.6K_1%_0402:35
- Flush:109: RES-1.6K_1%_0402:31 ↔ RES-1.6K_1%_0402:36
- [Flush]: RES-1.6K_1%_0402:38 ↔ RES-1.6K_1%_0402:39
- [Flush]: RES-1.6K_1%_0402:38 ↔ RES-1.6K_1%_0402:39
- [Flush]: RES-1.6K_1%_0402:40 ↔ RES-1.6K_1%_0402:42
- [Flush]: RES-1.6K_1%_0402:41 ↔ RES-1.6K_1%_0402:42
- [Flush]: RES-1.6K_1%_0402:40 ↔ RES-1.6K_1%_0402:41
- [Flush]: RES-1.6K_1%_0402:41 ↔ RES-1.6K_1%_0402:42
- [Flush]: RES-1.6K_1%_0402:39 ↔ RES-1.6K_1%_0402:41
- Flush:118: RES-1.6K_1%_0402:16 ↔ RES-1.6K_1%_0402:40
- Flush:119: C0603C101K5GAC3190:6 ↔ C0603C101K5GAC3190:7